# Autodesk Inventor assembly: Intake 2
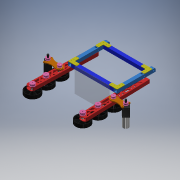
[picture p0: Inventor's stored thumbnail of the model, 180x180]
Saved by Autodesk Inventor 2017 SP1 (Build 210196100, 196)
## iProperties
Created: 2018-01-23
Part Number: Intake 2
Document SubType Name: Assembly
Designer: Ben
Mass: 3199.94 g
Surface Area: 15219.9 cm^2
Volume: 32265 cm^3
Density: 0.0991769 g/cm^3
Author: Ben
## Documents named in this file (13)
- C:\Users\Ben\Desktop\Projects\2018 Robot\Cube Intake\Intake 2.iam
- C:\Users\Ben\Desktop\Projects\2018 Robot\Cube Intake\arm.ipt
- C:\Users\Ben\Desktop\Projects\2018 Robot\Cube Intake\intake roller.ipt
- C:\Users\Ben\Desktop\Projects\2018 Robot\Cube Intake\pivot arm.ipt
- C:\Users\Ben\Desktop\Projects\2018 Robot\Cube Intake\cross brace.ipt
- C:\Users\Ben\Desktop\Projects\2018 Robot\Cube Intake\rest plate.ipt
- C:\Users\Ben\Desktop\Projects\2018 Robot\Cube Intake\micro cim.ipt
- C:\Users\Ben\Desktop\Projects\2018 Robot\Cube Intake\Part69.ipt
- C:\Users\Ben\Desktop\Projects\2018 Robot\Cube Intake\1277N450_CORROSION-RESISTANT TIMING BELT PULLEY.ipt
- C:\Users\Ben\Desktop\Projects\2018 Robot\Cube Intake\plate.ipt
- C:\Users\Ben\Desktop\Projects\2018 Robot\Cube Intake\Roller shaft.ipt
- C:\Users\Ben\Desktop\Projects\2018 Robot\Cube Intake\Roller drive shaft.ipt
- C:\Users\Ben\Desktop\Projects\2018 Robot\Cube Lift\18T XL Pulley.ipt
## Components (39 placed, 12 different names)
1. arm:1 — Symmetry:1, Insert:1, Insert:2, Insert:3, Insert:10, Insert:15, Insert:16, Insert:35, Insert:36, Insert:49, Insert:50, Insert:53
2. arm:2 — Symmetry:1, Insert:4, Insert:5, Insert:6, Insert:7, Insert:11, Insert:12, Insert:38, Insert:57, Insert:58, Insert:59
3. intake roller:1 — Insert:2, Insert:48
4. intake roller:2 — Insert:1
5. intake roller:3 — Insert:6, Insert:55
6. intake roller:4 — Insert:4, Insert:42
7. intake roller:5 — Insert:5, Insert:54
8. intake roller:6 — Insert:3, Insert:51
9. pivot arm:1 — Mate:6, Mate:7, Mate:8, Flush:3, Symmetry:2, Insert:7, Mate:16, Mate:17, Flush:8, Flush:9, Mate:18, Flush:10, Mate:20, Flush:15
10. pivot arm:2 — Mate:8, Flush:3, Symmetry:2, Angle:1, Flush:4, Flush:5, Mate:10, Insert:10, Mate:19, Flush:13, Mate:21, Flush:16
11. cross brace:1 — Flush:4, Flush:5, Mate:10, Mate:11, Flush:6, Mate:16, Flush:11, Flush:12
12. rest plate:1 — Mate:11, Flush:6, Flush:7
13. micro cim:1 — Insert:14, Insert:33, Mate:24
14. Part69:1 — Insert:11, Insert:12, Insert:14, Insert:33, Insert:56
15. Part69:2 — Insert:15, Insert:16, Insert:31, Insert:32, Mate:26, Insert:52
16. micro cim:2 — Insert:31, Insert:32, Mate:22
17. 1277N450_CORROSION-RESISTANT TIMING BELT PULLEY:1 — Mate:22, Mate:26
18. 1277N450_CORROSION-RESISTANT TIMING BELT PULLEY:4 — Insert:52
19. 1277N450_CORROSION-RESISTANT TIMING BELT PULLEY:5 — Mate:24
20. 1277N450_CORROSION-RESISTANT TIMING BELT PULLEY:6 — Insert:56
21. cross brace:2 — Mate:17, Flush:8, Flush:9, Flush:14, Flush:17
22. plate:1 — Mate:18, Flush:10, Flush:11
23. plate:2 — Mate:19, Flush:12, Flush:13
24. plate:3 — Mate:20, Flush:14, Flush:15
25. plate:4 — Mate:21, Flush:16, Flush:17
26. Roller shaft:1 — Insert:35
27. Roller drive shaft:1 — Insert:36
28. Roller shaft:2 — Insert:42
29. Roller drive shaft:2 — Insert:38
30. 18T XL Pulley:1 — Insert:55
31. 18T XL Pulley:2 — Insert:54
32. 18T XL Pulley:3 — Insert:57
33. 18T XL Pulley:4 — Insert:58
34. 18T XL Pulley:5 — Insert:51
35. 18T XL Pulley:6 — Insert:48
36. 18T XL Pulley:7 — Insert:50
37. 18T XL Pulley:8 — Insert:49
38. Roller drive shaft:3 — Insert:53
39. Roller drive shaft:4 — Insert:59
## Relationships (64: Insert 32, Flush 15, Mate 14, Symmetry 2, Angle 1)
- Symmetry:1: arm:1 ↔ arm:2
- Insert:1 (1.5875 mm): arm:1 ↔ intake roller:2
- Insert:2 (1.5875 mm): arm:1 ↔ intake roller:1
- Insert:3 (1.5875 mm): arm:1 ↔ intake roller:6
- Insert:4 (1.5875 mm): arm:2 ↔ intake roller:4
- Insert:5 (1.5875 mm): arm:2 ↔ intake roller:5
- Insert:6 (1.5875 mm): arm:2 ↔ intake roller:3
- Mate:6: pivot arm:1
- Mate:7: pivot arm:1
- Mate:8: pivot arm:1 ↔ pivot arm:2
- Flush:3: pivot arm:1 ↔ pivot arm:2
- Symmetry:2: pivot arm:1 ↔ pivot arm:2
- Insert:7 (1.5875 mm): arm:2 ↔ pivot arm:1
- Angle:1 (0 deg): pivot arm:2
- Flush:4: pivot arm:2 ↔ cross brace:1
- Flush:5: pivot arm:2 ↔ cross brace:1
- Mate:10: pivot arm:2 ↔ cross brace:1
- Mate:11: cross brace:1 ↔ rest plate:1
- Flush:6: cross brace:1 ↔ rest plate:1
- Flush:7: rest plate:1
- Mate:16: pivot arm:1 ↔ cross brace:1
- Insert:10 (1.5875 mm): arm:1 ↔ pivot arm:2
- Insert:11: arm:2 ↔ Part69:1
- Insert:12: arm:2 ↔ Part69:1
- Insert:14: micro cim:1 ↔ Part69:1
- Insert:15: arm:1 ↔ Part69:2
- Insert:16: arm:1 ↔ Part69:2
- Mate:17: pivot arm:1 ↔ cross brace:2
- Flush:8: pivot arm:1 ↔ cross brace:2
- Flush:9 (22.225 mm): pivot arm:1 ↔ cross brace:2
- Mate:18: pivot arm:1 ↔ plate:1
- Flush:10: pivot arm:1 ↔ plate:1
- Flush:11: cross brace:1 ↔ plate:1
- Mate:19: pivot arm:2 ↔ plate:2
- Flush:12: cross brace:1 ↔ plate:2
- Flush:13: pivot arm:2 ↔ plate:2
- Mate:20: pivot arm:1 ↔ plate:3
- Flush:14: cross brace:2 ↔ plate:3
- Flush:15: pivot arm:1 ↔ plate:3
- Mate:21: pivot arm:2 ↔ plate:4
- Flush:16: pivot arm:2 ↔ plate:4
- Flush:17: cross brace:2 ↔ plate:4
- Insert:31: Part69:2 ↔ micro cim:2
- Insert:32: Part69:2 ↔ micro cim:2
- Mate:22: micro cim:2 ↔ 1277N450_CORROSION-RESISTANT TIMING BELT PULLEY:1
- Insert:33: micro cim:1 ↔ Part69:1
- Mate:24: micro cim:1 ↔ 1277N450_CORROSION-RESISTANT TIMING BELT PULLEY:5
- Insert:35 (1.5875 mm): arm:1 ↔ Roller shaft:1
- Insert:36 (1.5875 mm): arm:1 ↔ Roller drive shaft:1
- Insert:38 (1.5875 mm): arm:2 ↔ Roller drive shaft:2
- Insert:42: intake roller:4 ↔ Roller shaft:2
- Insert:48: intake roller:1 ↔ 18T XL Pulley:6
- Insert:49 (1.5875 mm): arm:1 ↔ 18T XL Pulley:8
- Insert:50 (1.5875 mm): arm:1 ↔ 18T XL Pulley:7
- Insert:51: intake roller:6 ↔ 18T XL Pulley:5
- Mate:26 (1.5875 mm): Part69:2 ↔ 1277N450_CORROSION-RESISTANT TIMING BELT PULLEY:1
- Insert:52 (1.5875 mm): Part69:2 ↔ 1277N450_CORROSION-RESISTANT TIMING BELT PULLEY:4
- Insert:53 (1.5875 mm): arm:1 ↔ Roller drive shaft:3
- Insert:54: intake roller:5 ↔ 18T XL Pulley:2
- Insert:55: intake roller:3 ↔ 18T XL Pulley:1
- Insert:56 (1.5875 mm): Part69:1 ↔ 1277N450_CORROSION-RESISTANT TIMING BELT PULLEY:6
- Insert:57 (1.5875 mm): arm:2 ↔ 18T XL Pulley:3
- Insert:58 (1.5875 mm): arm:2 ↔ 18T XL Pulley:4
- Insert:59 (1.5875 mm): arm:2 ↔ Roller drive shaft:4
